# Autodesk Inventor assembly: 100-10-FRAME-DIFFERENTIAL-01
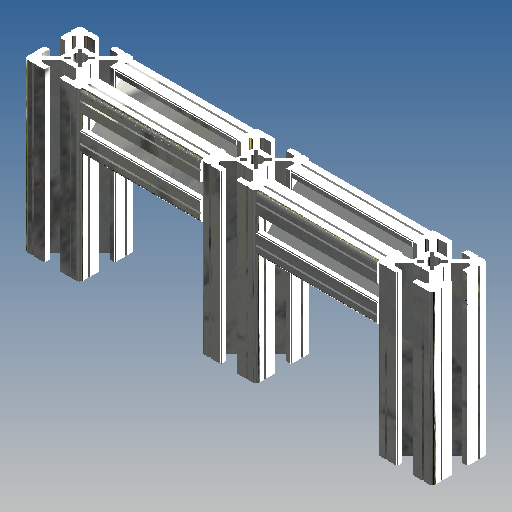
[picture p0: Inventor's stored thumbnail of the model, 512x512]
Saved by Autodesk Inventor 2018.2 (Build 222227000, 227)
## iProperties
Manager: feesmrt
Company: FRANCOR
Part Number: 100-10-FRAME-DIFFERENTIAL-01
Project: Rescue Robot
Cost Center: -
Material: Generisch
Document SubType Name: Assembly
Designer: feesmrt
Engineer: feesmrt
Authority: feesmrt
Description: Differential Profile Setup
Stock Number: 100-10-FRAME-DIFFERENTIAL-01
Subject: Rescue Robot
Author: feesmrt
Revision Number: 1
Title: Differential Profile Setup
## Documents named in this file (3)
- D:\Programmierung\FRANC0R\CAD\02-Rocker-Bogie-Robot\100-CHASSIS\10-FRAME\100-10-FRAME-DIFFERENTIAL-01.iam
- D:\Programmierung\FRANC0R\CAD\02-Rocker-Bogie-Robot\100-CHASSIS\10-FRAME\100-10-FRAME-PROFILE-DIFFERENTIAL-H.ipt
- D:\Programmierung\FRANC0R\CAD\02-Rocker-Bogie-Robot\100-CHASSIS\10-FRAME\100-10-FRAME-PROFILE-DIFFERENTIAL-W.ipt
## Components (5 placed, 2 different names)
1. 100-10-FRAME-PROFILE-DIFFERENTIAL-H:1 — Passend:1, Passend:2, Fluchtend:1, Passend:3, Passend:4, Fluchtend:2, Fluchtend:3, Fluchtend:4, Fluchtend:5
2. 100-10-FRAME-PROFILE-DIFFERENTIAL-H:2 — Passend:5, Passend:6, Fluchtend:6
3. 100-10-FRAME-PROFILE-DIFFERENTIAL-H:3 — Passend:7, Passend:8, Fluchtend:7
4. 100-10-FRAME-PROFILE-DIFFERENTIAL-W:1 — Passend:3, Fluchtend:3, Fluchtend:4, Passend:5, Passend:6, Fluchtend:6
5. 100-10-FRAME-PROFILE-DIFFERENTIAL-W:2 — Passend:4, Fluchtend:2, Fluchtend:5, Passend:7, Passend:8, Fluchtend:7
## Relationships (15: Mate 8, Flush 7)
- Passend:1 [Mate]: 100-10-FRAME-PROFILE-DIFFERENTIAL-H:1
- Passend:2 [Mate]: 100-10-FRAME-PROFILE-DIFFERENTIAL-H:1
- Fluchtend:1 [Flush]: 100-10-FRAME-PROFILE-DIFFERENTIAL-H:1
- Passend:3 [Mate]: 100-10-FRAME-PROFILE-DIFFERENTIAL-H:1 ↔ 100-10-FRAME-PROFILE-DIFFERENTIAL-W:1
- Passend:4 [Mate]: 100-10-FRAME-PROFILE-DIFFERENTIAL-H:1 ↔ 100-10-FRAME-PROFILE-DIFFERENTIAL-W:2
- Fluchtend:2 [Flush]: 100-10-FRAME-PROFILE-DIFFERENTIAL-H:1 ↔ 100-10-FRAME-PROFILE-DIFFERENTIAL-W:2
- Fluchtend:3 [Flush]: 100-10-FRAME-PROFILE-DIFFERENTIAL-H:1 ↔ 100-10-FRAME-PROFILE-DIFFERENTIAL-W:1
- Fluchtend:4 [Flush]: 100-10-FRAME-PROFILE-DIFFERENTIAL-H:1 ↔ 100-10-FRAME-PROFILE-DIFFERENTIAL-W:1
- Fluchtend:5 [Flush]: 100-10-FRAME-PROFILE-DIFFERENTIAL-H:1 ↔ 100-10-FRAME-PROFILE-DIFFERENTIAL-W:2
- Passend:5 [Mate]: 100-10-FRAME-PROFILE-DIFFERENTIAL-H:2 ↔ 100-10-FRAME-PROFILE-DIFFERENTIAL-W:1
- Passend:6 [Mate]: 100-10-FRAME-PROFILE-DIFFERENTIAL-H:2 ↔ 100-10-FRAME-PROFILE-DIFFERENTIAL-W:1
- Fluchtend:6 [Flush]: 100-10-FRAME-PROFILE-DIFFERENTIAL-H:2 ↔ 100-10-FRAME-PROFILE-DIFFERENTIAL-W:1
- Passend:7 [Mate]: 100-10-FRAME-PROFILE-DIFFERENTIAL-H:3 ↔ 100-10-FRAME-PROFILE-DIFFERENTIAL-W:2
- Passend:8 [Mate]: 100-10-FRAME-PROFILE-DIFFERENTIAL-H:3 ↔ 100-10-FRAME-PROFILE-DIFFERENTIAL-W:2
- Fluchtend:7 [Flush]: 100-10-FRAME-PROFILE-DIFFERENTIAL-H:3 ↔ 100-10-FRAME-PROFILE-DIFFERENTIAL-W:2
